# Autodesk Inventor assembly: Coil Designs
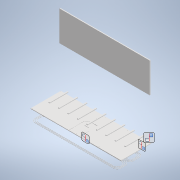
[picture p0: Inventor's stored thumbnail of the model, 180x180]
Saved by Autodesk Inventor 2021 (Build 250183000, 183)
## iProperties
Created: 2022-01-19
Part Number: Coil Designs
Document SubType Name: Assembly
Designer: avan411
Author: avan411
## Documents named in this file (6)
- H:\GitRepos\2021_SRW_RC_CAR\Magnetics\Tested coil designs\DoubleD\CadModels\Coil Designs.iam
- H:\GitRepos\2021_SRW_RC_CAR\Magnetics\Tested coil designs\DoubleD\CadModels\FerriteBar.ipt
- H:\GitRepos\2021_SRW_RC_CAR\Magnetics\Tested coil designs\DoubleD\CadModels\Part2.ipt
- H:\GitRepos\2021_SRW_RC_CAR\Magnetics\Tested coil designs\DoubleD\CadModels\coil.ipt
- H:\GitRepos\2021_SRW_RC_CAR\Magnetics\Tested coil designs\DoubleD\CadModels\PrimaryCoilFerriteLayer.ipt
- \\unifiles.uoa.auckland.ac.nz\myhome\Documents\btwnFerriteAndCoil.ipt
## Components (22 placed, 5 different names)
1. PrimaryCoilLayer:1 — Mate:5, Flush:1
2. coil:1
3. PrimaryCoiAluminiumlLayer:1
4. btwnFerriteAndCoil:1 — Flush:1
5. FerriteBar:2 — Mate:1, Mate:2
6. FerriteBar:1 — Mate:1, Mate:2
7. FerriteBar:3
8. FerriteBar:4
9. FerriteBar:5
10. FerriteBar:6
11. FerriteBar:7
12. FerriteBar:8
13. FerriteBar:9
14. FerriteBar:10
15. FerriteBar:11
16. FerriteBar:12
17. FerriteBar:13
18. FerriteBar:14
19. FerriteBar:15
20. FerriteBar:16
21. FerriteBar:17
22. FerriteBar:18 — Mate:5
## Component patterns: (9 elements, first: FerriteBar:2 + FerriteBar:1)
## Relationships (4: Mate 3, Flush 1)
- Mate:1: FerriteBar:2 ↔ FerriteBar:1
- Mate:2: FerriteBar:2 ↔ FerriteBar:1
- Mate:5 (41.6 mm): PrimaryCoilLayer:1 ↔ FerriteBar:18
- Flush:1: PrimaryCoilLayer:1 ↔ btwnFerriteAndCoil:1
